# Autodesk Inventor assembly: Lensfree_flexstage_box
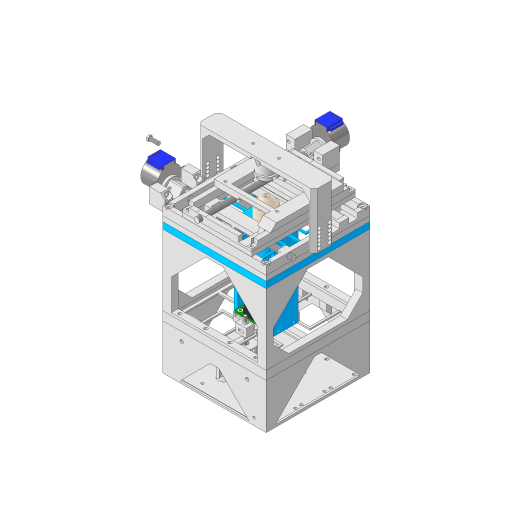
[picture p0: Inventor's stored thumbnail of the model, 512x512]
Saved by Autodesk Inventor 2023 (Build 270158000, 158)
## iProperties
Created: 2020-12-08
Part Number: Lensfree_flexstage_box
Document SubType Name: Assembly
Designer: CDT
Author: CDT
## Documents named in this file (30)
- C:\Users\CDT\Desktop\AutomatedSmartphoneMicroscopeForDiagnosisOfHelminths\CAD models\42. Smartphone_inverted_small_v9\Lensfree_flexstage_box.iam
- C:\Users\CDT\Desktop\AutomatedSmartphoneMicroscopeForDiagnosisOfHelminths\CAD models\42. Smartphone_inverted_small_v9\28BYJ-48 Stepper.ipt
- C:\Users\CDT\Desktop\AutomatedSmartphoneMicroscopeForDiagnosisOfHelminths\CAD models\42. Smartphone_inverted_small_v9\Bottom_carriage.ipt
- C:\Users\CDT\Desktop\AutomatedSmartphoneMicroscopeForDiagnosisOfHelminths\CAD models\42. Smartphone_inverted_small_v9\ULN2003 Stepper Driver.ipt
- C:\Users\CDT\Desktop\AutomatedSmartphoneMicroscopeForDiagnosisOfHelminths\CAD models\42. Smartphone_inverted_small_v9\160mm_shunt_box.ipt
- C:\Users\CDT\Desktop\AutomatedSmartphoneMicroscopeForDiagnosisOfHelminths\CAD models\42. Smartphone_inverted_small_v9\Raspberry Pi HQ Camera.ipt
- C:\Users\CDT\Desktop\AutomatedSmartphoneMicroscopeForDiagnosisOfHelminths\CAD models\42. Smartphone_inverted_small_v9\AC127-075-A-Step.ipt
- C:\Users\CDT\Desktop\AutomatedSmartphoneMicroscopeForDiagnosisOfHelminths\CAD models\42. Smartphone_inverted_small_v9\Flexible_tube_bolster_fixed_v3.ipt
- C:\Users\CDT\Desktop\AutomatedSmartphoneMicroscopeForDiagnosisOfHelminths\CAD models\42. Smartphone_inverted_small_v9\Objective_placeholder_V2.ipt
- C:\Users\CDT\Desktop\AutomatedSmartphoneMicroscopeForDiagnosisOfHelminths\CAD models\42. Smartphone_inverted_small_v9\slide_clips_4mm.ipt
- C:\Users\CDT\Desktop\AutomatedSmartphoneMicroscopeForDiagnosisOfHelminths\CAD models\42. Smartphone_inverted_small_v9\Flexible_cam_holder_v7_HQ.ipt
- C:\Users\CDT\Desktop\AutomatedSmartphoneMicroscopeForDiagnosisOfHelminths\CAD models\42. Smartphone_inverted_small_v9\RapberryPiZero.ipt
- C:\Users\CDT\Desktop\AutomatedSmartphoneMicroscopeForDiagnosisOfHelminths\CAD models\42. Smartphone_inverted_small_v9\Tube_lens_holder.ipt
- C:\Users\CDT\Desktop\AutomatedSmartphoneMicroscopeForDiagnosisOfHelminths\CAD models\42. Smartphone_inverted_small_v9\3mm_shaft_couple_sideclip_v4.ipt
- C:\Users\CDT\Desktop\AutomatedSmartphoneMicroscopeForDiagnosisOfHelminths\CAD models\42. Smartphone_inverted_small_v9\6mm_shaft_couple_sideclip_v2.ipt
- C:\Users\CDT\Desktop\AutomatedSmartphoneMicroscopeForDiagnosisOfHelminths\CAD models\42. Smartphone_inverted_small_v9\Rail_stage_x_m6_v2.ipt
- C:\Users\CDT\Desktop\AutomatedSmartphoneMicroscopeForDiagnosisOfHelminths\CAD models\42. Smartphone_inverted_small_v9\Rail_carriage_v2.ipt
- C:\Users\CDT\Desktop\AutomatedSmartphoneMicroscopeForDiagnosisOfHelminths\CAD models\42. Smartphone_inverted_small_v9\Rail_stage_y_v1.ipt
- C:\Users\CDT\Desktop\AutomatedSmartphoneMicroscopeForDiagnosisOfHelminths\CAD models\42. Smartphone_inverted_small_v9\Led_frame_2_4mm.ipt
- C:\Users\CDT\Desktop\AutomatedSmartphoneMicroscopeForDiagnosisOfHelminths\CAD models\42. Smartphone_inverted_small_v9\Rail_carriage_y_top_v2.ipt
- C:\Users\CDT\Desktop\AutomatedSmartphoneMicroscopeForDiagnosisOfHelminths\CAD models\42. Smartphone_inverted_small_v9\Stage_shunt.ipt
- C:\Users\CDT\Desktop\AutomatedSmartphoneMicroscopeForDiagnosisOfHelminths\CAD models\42. Smartphone_inverted_small_v9\M6 Screw.ipt
- C:\Users\CDT\Desktop\AutomatedSmartphoneMicroscopeForDiagnosisOfHelminths\CAD models\42. Smartphone_inverted_small_v9\stls\M3 screw.ipt
- C:\Users\CDT\Desktop\AutomatedSmartphoneMicroscopeForDiagnosisOfHelminths\CAD models\42. Smartphone_inverted_small_v9\stls\M3_nut.ipt
- C:\Users\CDT\Desktop\AutomatedSmartphoneMicroscopeForDiagnosisOfHelminths\CAD models\42. Smartphone_inverted_small_v9\stls\M3 nut.ipt
- C:\Users\CDT\Desktop\AutomatedSmartphoneMicroscopeForDiagnosisOfHelminths\CAD models\42. Smartphone_inverted_small_v9\stls\M4 bolt.ipt
- C:\Users\CDT\Desktop\AutomatedSmartphoneMicroscopeForDiagnosisOfHelminths\CAD models\42. Smartphone_inverted_small_v9\stls\m2.5.ipt
- C:\Users\CDT\Desktop\AutomatedSmartphoneMicroscopeForDiagnosisOfHelminths\CAD models\42. Smartphone_inverted_small_v9\stls\M3 screw_6mm.ipt
- C:\Users\CDT\Desktop\AutomatedSmartphoneMicroscopeForDiagnosisOfHelminths\CAD models\42. Smartphone_inverted_small_v9\1W_star_LED.ipt
- C:\Users\CDT\Desktop\AutomatedSmartphoneMicroscopeForDiagnosisOfHelminths\CAD models\42. Smartphone_inverted_small_v9\Condenser_holder_frame.ipt
## Components (41 placed, 29 different names)
1. M3 screw_6mm:2 — Mate:449
2. M3 screw_6mm:3 — Mate:456, Mate:457
3. M4 bolt:3 — Mate:459
4. 28BYJ-48 Stepper:7 — Mate:430, Mate:431, Mate:432, Mate:437
5. 28BYJ-48 Stepper:8 — Mate:427, Mate:428, Mate:429, Mate:436
6. Tube_lens_holder:1 — Mate:283, Mate:295, Mate:307
7. Objective_placeholder_V2:1 — Mate:238, Mate:287
8. Flexible_tube_bolster_fixed_v3:1 — Mate:238, Mate:239, Mate:283, Mate:287, Flush:92, Mate:288, Mate:295, Flush:127, Flush:128, Flush:129, Mate:447
9. Raspberry Pi HQ Camera:2 — Mate:420, Mate:421, Mate:422, Flush:136
10. AC127-075-A-Step:1 — Mate:239, Mate:307
11. 160mm_shunt_box:1 — Flush:92, Mate:288, Flush:127, Mate:423, Mate:424, Flush:130, Mate:426, Mate:445, Mate:446
12. 1W_star_LED:1 — Mate:451, Mate:452
13. M4 bolt:2 — Mate:448
14. M3 screw_6mm:1 — Mate:447
15. M3 nut:1
16. M4 bolt:1 — Mate:445, Mate:446
17. m2.5:1 — Flush:136
18. M3_nut:1 — Flush:134, Flush:135
19. M3 screw:2 — Mate:443
20. M3 screw:3 — Mate:444
21. 28BYJ-48 Stepper:9 — Mate:297, Mate:298, Mate:299, Mate:349, Mate:350, Mate:351, Mate:352
22. RapberryPiZero:1 — Mate:303, Mate:304, Mate:305
23. ULN2003 Stepper Driver:2 — Mate:61, Mate:62, Mate:63
24. ULN2003 Stepper Driver:3 — Mate:66, Mate:117
25. ULN2003 Stepper Driver:1 — Mate:58, Mate:72, Mate:73
26. Condenser_holder_frame:1 — Mate:453, Mate:454, Mate:455, Mate:456, Mate:457
27. M3 screw:1 — Flush:133, Flush:134, Flush:135
28. M6 Screw:1 — Mate:439, Mate:440
29. M6 Screw:2 — Mate:441, Mate:442
30. 6mm_shaft_couple_sideclip_v2:2 — Mate:437, Mate:438, Mate:442
31. Stage_shunt:1 — Flush:128, Flush:129, Flush:130, Mate:425, Flush:131, Flush:132
32. Rail_carriage_y_top_v2:1 — Flush:124, Mate:419
33. Rail_carriage_v2:1 — Mate:412, Flush:118, Flush:120, Mate:414, Flush:121
34. Rail_stage_x_m6_v2:1 — Mate:412, Flush:118, Mate:425, Flush:131, Flush:132, Mate:427, Mate:428, Mate:429, Mate:433, Mate:434, Mate:435, Mate:440, Mate:448, Mate:450
35. Rail_stage_y_v1:1 — Flush:120, Mate:414, Flush:121, Flush:124, Mate:419, Mate:430, Mate:431, Mate:432, Mate:438, Mate:441, Mate:449
36. Led_frame_2_4mm:1 — Mate:433, Mate:434, Mate:450, Mate:451, Mate:452, Mate:453, Mate:454, Mate:455, Mate:459
37. 6mm_shaft_couple_sideclip_v2:1 — Mate:435, Mate:436, Mate:439
38. 3mm_shaft_couple_sideclip_v4:2 — Mate:349, Mate:350, Mate:352, Flush:133, Mate:443, Mate:444
39. Flexible_cam_holder_v7_HQ:2 — Flush:108, Flush:109, Mate:364, Mate:420, Mate:421, Mate:422, Mate:423, Mate:424, Mate:426
40. slide_clips_4mm:1
41. Bottom_carriage:1 — Mate:58, Mate:61, Mate:62, Mate:63, Mate:66, Mate:72, Mate:73, Mate:117, Mate:297, Mate:298, Mate:299, Mate:303, Mate:304, Mate:305, Mate:351, Flush:108, Flush:109, Mate:364
## Relationships (85: Mate 68, Flush 17)
- Mate:58 (1 mm): ULN2003 Stepper Driver:1 ↔ Bottom_carriage:1
- Mate:61: ULN2003 Stepper Driver:2 ↔ Bottom_carriage:1
- Mate:62: ULN2003 Stepper Driver:2 ↔ Bottom_carriage:1
- Mate:63: ULN2003 Stepper Driver:2 ↔ Bottom_carriage:1
- Mate:66: ULN2003 Stepper Driver:3 ↔ Bottom_carriage:1
- Mate:72: ULN2003 Stepper Driver:1 ↔ Bottom_carriage:1
- Mate:73: ULN2003 Stepper Driver:1 ↔ Bottom_carriage:1
- Mate:117: ULN2003 Stepper Driver:3 ↔ Bottom_carriage:1
- Mate:238: Objective_placeholder_V2:1 ↔ Flexible_tube_bolster_fixed_v3:1
- Mate:239: Flexible_tube_bolster_fixed_v3:1 ↔ AC127-075-A-Step:1
- Mate:283: Tube_lens_holder:1 ↔ Flexible_tube_bolster_fixed_v3:1
- Mate:287: Objective_placeholder_V2:1 ↔ Flexible_tube_bolster_fixed_v3:1
- Flush:92: Flexible_tube_bolster_fixed_v3:1 ↔ 160mm_shunt_box:1
- Mate:288: Flexible_tube_bolster_fixed_v3:1 ↔ 160mm_shunt_box:1
- Mate:295 (60 mm): Tube_lens_holder:1 ↔ Flexible_tube_bolster_fixed_v3:1
- Mate:297: 28BYJ-48 Stepper:9 ↔ Bottom_carriage:1
- Mate:298: 28BYJ-48 Stepper:9 ↔ Bottom_carriage:1
- Mate:299: 28BYJ-48 Stepper:9 ↔ Bottom_carriage:1
- Mate:303: RapberryPiZero:1 ↔ Bottom_carriage:1
- Mate:304: RapberryPiZero:1 ↔ Bottom_carriage:1
- Mate:305: RapberryPiZero:1 ↔ Bottom_carriage:1
- Mate:307 (-120 mm): Tube_lens_holder:1 ↔ AC127-075-A-Step:1
- Mate:349: 28BYJ-48 Stepper:9 ↔ 3mm_shaft_couple_sideclip_v4:2
- Mate:350: 28BYJ-48 Stepper:9 ↔ 3mm_shaft_couple_sideclip_v4:2
- Mate:351: 28BYJ-48 Stepper:9 ↔ Bottom_carriage:1
- Mate:352: 28BYJ-48 Stepper:9 ↔ 3mm_shaft_couple_sideclip_v4:2
- Flush:108: Flexible_cam_holder_v7_HQ:2 ↔ Bottom_carriage:1
- Flush:109: Flexible_cam_holder_v7_HQ:2 ↔ Bottom_carriage:1
- Mate:364: Flexible_cam_holder_v7_HQ:2 ↔ Bottom_carriage:1
- Mate:412 (0.1 mm): Rail_carriage_v2:1 ↔ Rail_stage_x_m6_v2:1
- Flush:118: Rail_carriage_v2:1 ↔ Rail_stage_x_m6_v2:1
- Flush:120: Rail_carriage_v2:1 ↔ Rail_stage_y_v1:1
- Mate:414: Rail_carriage_v2:1 ↔ Rail_stage_y_v1:1
- Flush:121: Rail_carriage_v2:1 ↔ Rail_stage_y_v1:1
- Flush:124: Rail_carriage_y_top_v2:1 ↔ Rail_stage_y_v1:1
- Mate:419: Rail_carriage_y_top_v2:1 ↔ Rail_stage_y_v1:1
- Mate:420: Raspberry Pi HQ Camera:2 ↔ Flexible_cam_holder_v7_HQ:2
- Mate:421: Raspberry Pi HQ Camera:2 ↔ Flexible_cam_holder_v7_HQ:2
- Mate:422: Raspberry Pi HQ Camera:2 ↔ Flexible_cam_holder_v7_HQ:2
- Flush:127: Flexible_tube_bolster_fixed_v3:1 ↔ 160mm_shunt_box:1
- Flush:128: Flexible_tube_bolster_fixed_v3:1 ↔ Stage_shunt:1
- Mate:423: 160mm_shunt_box:1 ↔ Flexible_cam_holder_v7_HQ:2
- Mate:424: 160mm_shunt_box:1 ↔ Flexible_cam_holder_v7_HQ:2
- Flush:129: Flexible_tube_bolster_fixed_v3:1 ↔ Stage_shunt:1
- Flush:130: 160mm_shunt_box:1 ↔ Stage_shunt:1
- Mate:425: Stage_shunt:1 ↔ Rail_stage_x_m6_v2:1
- Flush:131: Stage_shunt:1 ↔ Rail_stage_x_m6_v2:1
- Mate:426: 160mm_shunt_box:1 ↔ Flexible_cam_holder_v7_HQ:2
- Flush:132: Stage_shunt:1 ↔ Rail_stage_x_m6_v2:1
- Mate:427: 28BYJ-48 Stepper:8 ↔ Rail_stage_x_m6_v2:1
- Mate:428: 28BYJ-48 Stepper:8 ↔ Rail_stage_x_m6_v2:1
- Mate:429: 28BYJ-48 Stepper:8 ↔ Rail_stage_x_m6_v2:1
- Mate:430: 28BYJ-48 Stepper:7 ↔ Rail_stage_y_v1:1
- Mate:431: 28BYJ-48 Stepper:7 ↔ Rail_stage_y_v1:1
- Mate:432: 28BYJ-48 Stepper:7 ↔ Rail_stage_y_v1:1
- Mate:433: Rail_stage_x_m6_v2:1 ↔ Led_frame_2_4mm:1
- Mate:434: Rail_stage_x_m6_v2:1 ↔ Led_frame_2_4mm:1
- Mate:435: Rail_stage_x_m6_v2:1 ↔ 6mm_shaft_couple_sideclip_v2:1
- Mate:436: 28BYJ-48 Stepper:8 ↔ 6mm_shaft_couple_sideclip_v2:1
- Mate:437: 28BYJ-48 Stepper:7 ↔ 6mm_shaft_couple_sideclip_v2:2
- Mate:438: 6mm_shaft_couple_sideclip_v2:2 ↔ Rail_stage_y_v1:1
- Mate:439: M6 Screw:1 ↔ 6mm_shaft_couple_sideclip_v2:1
- Mate:440: M6 Screw:1 ↔ Rail_stage_x_m6_v2:1
- Mate:441: M6 Screw:2 ↔ Rail_stage_y_v1:1
- Mate:442: M6 Screw:2 ↔ 6mm_shaft_couple_sideclip_v2:2
- Flush:133: M3 screw:1 ↔ 3mm_shaft_couple_sideclip_v4:2
- Flush:134: M3_nut:1 ↔ M3 screw:1
- Flush:135: M3_nut:1 ↔ M3 screw:1
- Mate:443: M3 screw:2 ↔ 3mm_shaft_couple_sideclip_v4:2
- Mate:444: M3 screw:3 ↔ 3mm_shaft_couple_sideclip_v4:2
- Mate:445 (60 mm): 160mm_shunt_box:1 ↔ M4 bolt:1
- Mate:446: 160mm_shunt_box:1 ↔ M4 bolt:1
- Flush:136 (80 mm): Raspberry Pi HQ Camera:2 ↔ m2.5:1
- Mate:447: Flexible_tube_bolster_fixed_v3:1 ↔ M3 screw_6mm:1
- Mate:448: M4 bolt:2 ↔ Rail_stage_x_m6_v2:1
- Mate:449: M3 screw_6mm:2 ↔ Rail_stage_y_v1:1
- Mate:450: Rail_stage_x_m6_v2:1 ↔ Led_frame_2_4mm:1
- Mate:451: 1W_star_LED:1 ↔ Led_frame_2_4mm:1
- Mate:452: 1W_star_LED:1 ↔ Led_frame_2_4mm:1
- Mate:453: Condenser_holder_frame:1 ↔ Led_frame_2_4mm:1
- Mate:454: Condenser_holder_frame:1 ↔ Led_frame_2_4mm:1
- Mate:455: Condenser_holder_frame:1 ↔ Led_frame_2_4mm:1
- Mate:456: M3 screw_6mm:3 ↔ Condenser_holder_frame:1
- Mate:457 (20 mm): M3 screw_6mm:3 ↔ Condenser_holder_frame:1
- Mate:459: M4 bolt:3 ↔ Led_frame_2_4mm:1
